# Autodesk Inventor assembly: tau2
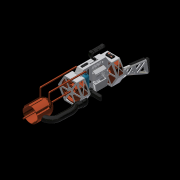
[picture p0: Inventor's stored thumbnail of the model, 180x180]
Saved by Autodesk Inventor 2020.4 (Build 244396010, 396A)
## iProperties
Created: 2022-09-08
Part Number: tau2
Document SubType Name: Assembly
Designer: Val
Author: Val
## Documents named in this file (37)
- C:\Users\Val\Desktop\tau\Tau.iam
- C:\Users\Val\Desktop\tau\external\TopHandle.ipt
- C:\Users\Val\Desktop\tau\Body.ipt
- C:\Users\Val\Desktop\tau\external\FlowMeter.ipt
- C:\Users\Val\Desktop\tau\external\SideHandle.ipt
- C:\Users\Val\Desktop\tau\external\SideHandleBase.ipt
- C:\Users\Val\Desktop\tau\HexCoil.ipt
- C:\Users\Val\Desktop\tau\CoilCover.ipt
- C:\Users\Val\Desktop\tau\Stock.ipt
- C:\Users\Val\Desktop\tau\Stock_MIR.ipt
- C:\Users\Val\Desktop\tau\HoseConnector.ipt
- C:\Users\Val\Desktop\tau\BatteryCover.ipt
- C:\Users\Val\Desktop\tau\BatteryCoverLid.ipt
- C:\Users\Val\Desktop\tau\MuzzleTube.ipt
- C:\Users\Val\Desktop\tau\TopPipe.ipt
- C:\Users\Val\Desktop\tau\external\CO2Cartridge16g.ipt
- C:\Users\Val\Desktop\tau\external\Picatinny6.ipt
- C:\Users\Val\Desktop\tau\BatteryHeatsink.ipt
- C:\Users\Val\Desktop\tau\BodyMirror.ipt
- C:\Users\Val\Desktop\tau\TopPipeStraight.ipt
- C:\Users\Val\Desktop\tau\BatteryPlate.ipt
- C:\Users\Val\Desktop\tau\StockBack.ipt
- C:\Users\Val\Desktop\tau\external\CO2FeedPipe.ipt
- C:\Users\Val\Desktop\tau\external\Picatinny10.ipt
- C:\Users\Val\Desktop\tau\external\Picatinny14.ipt
- C:\Users\Val\Desktop\tau\StockGrip.ipt
- C:\Users\Val\Desktop\tau\quote\TCap.ipt
- C:\Users\Val\Desktop\tau\quote\TCore.ipt
- C:\Users\Val\Documents\Inventor\Content Center Files\R2020\en-US\ANSI B18.3(05)\ANSI B18.3 - 7_16-20 UNF - 0.5(31).ipt
- C:\Users\Val\Documents\Inventor\Content Center Files\R2020\en-US\AS 1420\AS 1420 - 1973 - M5 x 10.ipt
- C:\Users\Val\Documents\Inventor\Content Center Files\R2020\en-US\ANSI B18.3(05)\ANSI B18.3 - 10-32 UNF - 0.25(31).ipt
- C:\Users\Val\Documents\Inventor\Content Center Files\R2020\en-US\ANSI B18.3(05)\ANSI B18.3 - 4-40 UNC - 0.1875(31).ipt
- C:\Users\Val\Desktop\tau\external\9600K72_SBR Rubber Grommet.ipt
- C:\Users\Val\Desktop\tau\quote\MEndTurned3.ipt
- C:\Users\Val\Desktop\tau\external\Batteries\2 x AA Battery Holder .iam
- C:\Users\Val\Desktop\tau\MFinal.ipt
- C:\Users\Val\Desktop\tau\external\TorDigikey.ipt
## Components (64 placed, 36 different names)
1. TopHandle:1 — Mate:160, Mate:161
2. Body:1 — Mate:1, Mate:3, Mate:4, Mate:6, Mate:15, Mate:26, Mate:30, Flush:35, Mate:37, Mate:38, Mate:56, Mate:79, Mate:80, Mate:81, Mate:98, Mate:100, Angle:7, Flush:48, Mate:103, Insert:1, Insert:2, Mate:117, Mate:119, Mate:121, Angle:9, Mate:144, Mate:161
3. FlowMeter:1 — Mate:3, Mate:4, Mate:6
4. SideHandle:1 — Mate:52, Mate:53
5. HexCoil:1 — Mate:13, Mate:15, Flush:6, Flush:7, Mate:27, Flush:10, Flush:11, Mate:31, Flush:12, Flush:13, Flush:37, Insert:9, Insert:10, Insert:11, Insert:12, Mate:141
6. HexCoil:2 — Flush:6, Flush:7, Mate:22, Flush:8, Mate:24, Flush:9, Mate:25, Flush:35, Insert:13, Insert:14, Insert:15, Insert:16, Mate:147, Mate:154, Mate:166
7. CoilCover:1 — Mate:22, Flush:8, Mate:25, Mate:113
8. CoilCover:2 — Mate:24, Flush:9, Mate:26, Mate:158
9. CoilCover:3 — Mate:31, Flush:12, Flush:13, Flush:36, Mate:33, Mate:142, Flush:52, Mate:151
10. CoilCover:4 — Mate:27, Flush:10, Flush:11, Mate:30
11. Stock:1 — Flush:34, Mate:105, Insert:4, Insert:5, Insert:6, Insert:7, Insert:8, Mate:145, Mate:150, Mate:154, Mate:155
12. Stock_MIR:1 — Mate:106, Mate:109, Mate:110, Mate:146, Mate:147, Mate:156
13. HoseConnector:1 — Flush:36, Mate:33, Flush:37
14. BatteryCover:1 — Flush:38, Flush:39, Flush:44, Flush:45, Mate:66, Mate:67, Mate:68, Mate:85, Mate:86, Mate:87
15. BatteryCover:2 — Flush:38, Mate:35, Flush:40, Flush:41, Mate:64, Mate:65, Angle:6, Mate:88, Mate:89, Mate:90
16. BatteryCover:3 — Flush:39, Mate:36, Flush:42, Flush:43, Mate:39, Flush:46, Flush:47, Mate:69, Mate:70, Mate:71, Mate:91, Mate:92, Mate:93
17. BatteryCoverLid:1 — Mate:35, Flush:40, Flush:41, Mate:36, Flush:42, Flush:43, Flush:44, Flush:45, Mate:37, Mate:38
18. BatteryCoverLid:2 — Mate:39, Flush:46, Flush:47
19. MuzzleTube:1 — Mate:116, Mate:142, Mate:167
20. TopPipe:1 — Mate:165, Flush:53
21. CO2Cartridge16g:1 — Mate:94, Mate:163
22. Picatinny6:2 — Mate:56, Mate:98, Mate:99, Mate:153
23. SideHandleBase:1 — Mate:52, Mate:53, Mate:107, Mate:108
24. BatteryHeatsink:1 — Mate:64, Mate:65, Angle:6, Mate:136, Mate:137
25. BatteryHeatsink:2 — Mate:66, Mate:67, Mate:68
26. BatteryHeatsink:3 — Mate:69, Mate:70, Mate:71
27. BodyMirror:1 — Mate:79, Mate:80, Mate:81, Mate:99, Mate:101, Angle:8, Flush:49, Mate:102, Flush:51, Mate:118, Mate:120, Mate:122, Mate:143, Mate:153, Mate:158, Mate:160, Mate:165
28. TopPipeStraight:1 — Mate:94, Angle:10, Mate:163, Flush:53
29. BatteryPlate:1 — Mate:85, Mate:86, Mate:87
30. BatteryPlate:2 — Mate:88, Mate:89, Mate:90
31. BatteryPlate:3 — Mate:91, Mate:92, Mate:93
32. StockBack:1 — Mate:150, Mate:155, Mate:156
33. CO2FeedPipe:1 — Mate:140, Mate:152
34. Picatinny10:1 — Mate:100, Angle:7, Flush:48, Flush:50, Mate:107, Mate:108, Mate:144
35. Picatinny10:2 — Mate:101, Angle:8, Flush:49, Flush:50
36. Picatinny14:1 — Mate:104, Mate:105, Mate:106
37. Picatinny10:3 — Mate:102, Mate:103, Flush:51
38. StockGrip:1 — Mate:109, Mate:110
39. TCap:1 — Mate:113, Mate:168
40. TCore:2 — Mate:116, Flush:52
41. Hexagon Socket Head Cap Screw - Inch 7/16-20 UNF - 0.5:1 — Insert:1
42. Hexagon Socket Head Cap Screw - Inch 7/16-20 UNF - 0.5:2 — Insert:2
43. Hexagon Socket Head Cap Screw - Inch 7/16-20 UNF - 0.5:4 — Mate:117, Mate:118
44. Hexagon Socket Head Cap Screw - Inch 7/16-20 UNF - 0.5:5 — Mate:119, Mate:120
45. Hexagon Socket Head Cap Screw - Inch 7/16-20 UNF - 0.5:6 — Mate:121, Mate:122
46. AS 1420 - Metric M5 x 10:1 — Insert:4
47. AS 1420 - Metric M5 x 10:2 — Insert:5
48. AS 1420 - Metric M5 x 10:3 — Insert:6
49. AS 1420 - Metric M5 x 10:4 — Insert:7
50. AS 1420 - Metric M5 x 10:5 — Insert:8
51. Hexagon Socket Head Cap Screw - Inch 10-32 UNF - 0.25:1 — Insert:9
52. Hexagon Socket Head Cap Screw - Inch 10-32 UNF - 0.25:2 — Insert:10
53. Hexagon Socket Head Cap Screw - Inch 10-32 UNF - 0.25:3 — Insert:11
54. Hexagon Socket Head Cap Screw - Inch 10-32 UNF - 0.25:4 — Insert:12
55. Hexagon Socket Head Cap Screw - Inch 10-32 UNF - 0.25:5 — Insert:13, Mate:146
56. Hexagon Socket Head Cap Screw - Inch 10-32 UNF - 0.25:6 — Insert:14, Mate:145
57. Hexagon Socket Head Cap Screw - Inch 10-32 UNF - 0.25:7 — Insert:15
58. Hexagon Socket Head Cap Screw - Inch 10-32 UNF - 0.25:8 — Insert:16
59. Hexagon Socket Head Cap Screw - Inch No. 4 - 40 UNC - 3/16:1 — Mate:136, Mate:137
60. MEndTurned3:1 — Angle:9
61. 9600K72_SBR Rubber Grommet:1 — Mate:140, Mate:152
62. 2 x AA Battery Holder :1 [sub-assembly] — Mate:166
63. MFinal:1 — Mate:167
64. TorDigikey:1 — Mate:168
## Relationships (138: Mate 89, Flush 28, Insert 15, Angle 5, Symmetry 1)
- Symmetry:1
- Mate:1: Body:1
- Mate:3: Body:1 ↔ FlowMeter:1
- Mate:4: Body:1 ↔ FlowMeter:1
- Mate:6: Body:1 ↔ FlowMeter:1
- Mate:13: HexCoil:1
- Mate:15: Body:1 ↔ HexCoil:1
- Flush:6: HexCoil:1 ↔ HexCoil:2
- Flush:7: HexCoil:1 ↔ HexCoil:2
- Mate:22: HexCoil:2 ↔ CoilCover:1
- Flush:8: HexCoil:2 ↔ CoilCover:1
- Mate:24: HexCoil:2 ↔ CoilCover:2
- Flush:9: HexCoil:2 ↔ CoilCover:2
- Mate:25: HexCoil:2 ↔ CoilCover:1
- Mate:26: Body:1 ↔ CoilCover:2
- Mate:27: HexCoil:1 ↔ CoilCover:4
- Flush:10: HexCoil:1 ↔ CoilCover:4
- Flush:11: HexCoil:1 ↔ CoilCover:4
- Mate:30: Body:1 ↔ CoilCover:4
- Mate:31: HexCoil:1 ↔ CoilCover:3
- Flush:12: HexCoil:1 ↔ CoilCover:3
- Flush:13: HexCoil:1 ↔ CoilCover:3
- Flush:34: Stock:1
- Flush:35: Body:1 ↔ HexCoil:2
- Flush:36: CoilCover:3 ↔ HoseConnector:1
- Mate:33: CoilCover:3 ↔ HoseConnector:1
- Flush:37: HexCoil:1 ↔ HoseConnector:1
- Flush:38: BatteryCover:1 ↔ BatteryCover:2
- Flush:39: BatteryCover:1 ↔ BatteryCover:3
- Mate:35: BatteryCover:2 ↔ BatteryCoverLid:1
- Flush:40: BatteryCover:2 ↔ BatteryCoverLid:1
- Flush:41: BatteryCover:2 ↔ BatteryCoverLid:1
- Mate:36: BatteryCover:3 ↔ BatteryCoverLid:1
- Flush:42: BatteryCover:3 ↔ BatteryCoverLid:1
- Flush:43: BatteryCover:3 ↔ BatteryCoverLid:1
- Flush:44: BatteryCover:1 ↔ BatteryCoverLid:1
- Flush:45: BatteryCover:1 ↔ BatteryCoverLid:1
- Mate:37: Body:1 ↔ BatteryCoverLid:1
- Mate:38: Body:1 ↔ BatteryCoverLid:1
- Mate:39: BatteryCover:3 ↔ BatteryCoverLid:2
- Flush:46: BatteryCover:3 ↔ BatteryCoverLid:2
- Flush:47: BatteryCover:3 ↔ BatteryCoverLid:2
- Mate:52: SideHandle:1 ↔ SideHandleBase:1
- Mate:53: SideHandle:1 ↔ SideHandleBase:1
- Mate:56: Body:1 ↔ Picatinny6:2
- Mate:64: BatteryCover:2 ↔ BatteryHeatsink:1
- Mate:65: BatteryCover:2 ↔ BatteryHeatsink:1
- Angle:6 (0 deg): BatteryCover:2 ↔ BatteryHeatsink:1
- Mate:66: BatteryCover:1 ↔ BatteryHeatsink:2
- Mate:67: BatteryCover:1 ↔ BatteryHeatsink:2
- Mate:68: BatteryCover:1 ↔ BatteryHeatsink:2
- Mate:69: BatteryCover:3 ↔ BatteryHeatsink:3
- Mate:70: BatteryCover:3 ↔ BatteryHeatsink:3
- Mate:71: BatteryCover:3 ↔ BatteryHeatsink:3
- Mate:79: Body:1 ↔ BodyMirror:1
- Mate:80: Body:1 ↔ BodyMirror:1
- Mate:81: Body:1 ↔ BodyMirror:1
- Mate:85: BatteryCover:1 ↔ BatteryPlate:1
- Mate:86: BatteryCover:1 ↔ BatteryPlate:1
- Mate:87: BatteryCover:1 ↔ BatteryPlate:1
- Mate:88: BatteryCover:2 ↔ BatteryPlate:2
- Mate:89: BatteryCover:2 ↔ BatteryPlate:2
- Mate:90: BatteryCover:2 ↔ BatteryPlate:2
- Mate:91: BatteryCover:3 ↔ BatteryPlate:3
- Mate:92: BatteryCover:3 ↔ BatteryPlate:3
- Mate:93: BatteryCover:3 ↔ BatteryPlate:3
- Mate:94: CO2Cartridge16g:1 ↔ TopPipeStraight:1
- Mate:98: Body:1 ↔ Picatinny6:2
- Mate:99 (8.4667 mm): Picatinny6:2 ↔ BodyMirror:1
- Mate:100: Body:1 ↔ Picatinny10:1
- Angle:7 (0 deg): Body:1 ↔ Picatinny10:1
- Flush:48 (-5 mm): Body:1 ↔ Picatinny10:1
- Mate:101: BodyMirror:1 ↔ Picatinny10:2
- Angle:8 (0 deg): BodyMirror:1 ↔ Picatinny10:2
- Flush:49 (5 mm): BodyMirror:1 ↔ Picatinny10:2
- Flush:50: Picatinny10:1 ↔ Picatinny10:2
- Mate:102: BodyMirror:1 ↔ Picatinny10:3
- Mate:103: Body:1 ↔ Picatinny10:3
- Flush:51 (-5 mm): BodyMirror:1 ↔ Picatinny10:3
- Mate:104: Picatinny14:1
- Mate:105: Stock:1 ↔ Picatinny14:1
- Mate:106 (6 mm): Stock_MIR:1 ↔ Picatinny14:1
- Mate:107: SideHandleBase:1 ↔ Picatinny10:1
- Mate:108: SideHandleBase:1 ↔ Picatinny10:1
- Mate:109: Stock_MIR:1 ↔ StockGrip:1
- Mate:110: Stock_MIR:1 ↔ StockGrip:1
- Mate:113: CoilCover:1 ↔ TCap:1
- Mate:116: MuzzleTube:1 ↔ TCore:2
- Insert:1: Body:1 ↔ Hexagon Socket Head Cap Screw - Inch 7/16-20 UNF - 0.5:1
- Insert:2: Body:1 ↔ Hexagon Socket Head Cap Screw - Inch 7/16-20 UNF - 0.5:2
- Mate:117: Body:1 ↔ Hexagon Socket Head Cap Screw - Inch 7/16-20 UNF - 0.5:4
- Mate:118: BodyMirror:1 ↔ Hexagon Socket Head Cap Screw - Inch 7/16-20 UNF - 0.5:4
- Mate:119: Body:1 ↔ Hexagon Socket Head Cap Screw - Inch 7/16-20 UNF - 0.5:5
- Mate:120: BodyMirror:1 ↔ Hexagon Socket Head Cap Screw - Inch 7/16-20 UNF - 0.5:5
- Mate:121: Body:1 ↔ Hexagon Socket Head Cap Screw - Inch 7/16-20 UNF - 0.5:6
- Mate:122: BodyMirror:1 ↔ Hexagon Socket Head Cap Screw - Inch 7/16-20 UNF - 0.5:6
- Insert:4: Stock:1 ↔ AS 1420 - Metric M5 x 10:1
- Insert:5: Stock:1 ↔ AS 1420 - Metric M5 x 10:2
- Insert:6: Stock:1 ↔ AS 1420 - Metric M5 x 10:3
- Insert:7: Stock:1 ↔ AS 1420 - Metric M5 x 10:4
- Insert:8: Stock:1 ↔ AS 1420 - Metric M5 x 10:5
- Insert:9: HexCoil:1 ↔ Hexagon Socket Head Cap Screw - Inch 10-32 UNF - 0.25:1
- Insert:10: HexCoil:1 ↔ Hexagon Socket Head Cap Screw - Inch 10-32 UNF - 0.25:2
- Insert:11: HexCoil:1 ↔ Hexagon Socket Head Cap Screw - Inch 10-32 UNF - 0.25:3
- Insert:12: HexCoil:1 ↔ Hexagon Socket Head Cap Screw - Inch 10-32 UNF - 0.25:4
- Insert:13: HexCoil:2 ↔ Hexagon Socket Head Cap Screw - Inch 10-32 UNF - 0.25:5
- Insert:14: HexCoil:2 ↔ Hexagon Socket Head Cap Screw - Inch 10-32 UNF - 0.25:6
- Insert:15: HexCoil:2 ↔ Hexagon Socket Head Cap Screw - Inch 10-32 UNF - 0.25:7
- Insert:16: HexCoil:2 ↔ Hexagon Socket Head Cap Screw - Inch 10-32 UNF - 0.25:8
- Mate:136: BatteryHeatsink:1 ↔ Hexagon Socket Head Cap Screw - Inch No. 4 - 40 UNC - 3/16:1
- Mate:137: BatteryHeatsink:1 ↔ Hexagon Socket Head Cap Screw - Inch No. 4 - 40 UNC - 3/16:1
- Angle:9 (0 deg): Body:1 ↔ MEndTurned3:1
- Mate:140: CO2FeedPipe:1 ↔ 9600K72_SBR Rubber Grommet:1
- Mate:141: HexCoil:1
- Mate:142: CoilCover:3 ↔ MuzzleTube:1
- Flush:52 (8.4582 mm): CoilCover:3 ↔ TCore:2
- Mate:143: BodyMirror:1
- Mate:144: Body:1 ↔ Picatinny10:1
- Mate:145: Stock:1 ↔ Hexagon Socket Head Cap Screw - Inch 10-32 UNF - 0.25:6
- Mate:146: Stock_MIR:1 ↔ Hexagon Socket Head Cap Screw - Inch 10-32 UNF - 0.25:5
- Mate:147: HexCoil:2 ↔ Stock_MIR:1
- Mate:150: Stock:1 ↔ StockBack:1
- Mate:151: CoilCover:3
- Mate:152: CO2FeedPipe:1 ↔ 9600K72_SBR Rubber Grommet:1
- Mate:153: Picatinny6:2 ↔ BodyMirror:1
- Mate:154: HexCoil:2 ↔ Stock:1
- Mate:155: Stock:1 ↔ StockBack:1
- Mate:156: Stock_MIR:1 ↔ StockBack:1
- Mate:158: CoilCover:2 ↔ BodyMirror:1
- Mate:160: TopHandle:1 ↔ BodyMirror:1
- Mate:161: TopHandle:1 ↔ Body:1
- Angle:10 (0 deg): TopPipeStraight:1
- Mate:163 (-12.7 mm): CO2Cartridge16g:1 ↔ TopPipeStraight:1
- Mate:165: TopPipe:1 ↔ BodyMirror:1
- Flush:53: TopPipe:1 ↔ TopPipeStraight:1
- Mate:166: HexCoil:2 ↔ 2 x AA Battery Holder :1
- Mate:167: MuzzleTube:1 ↔ MFinal:1
- Mate:168: TCap:1 ↔ TorDigikey:1
